# Autodesk Inventor assembly: rapoukMotherboardAssemblyv0
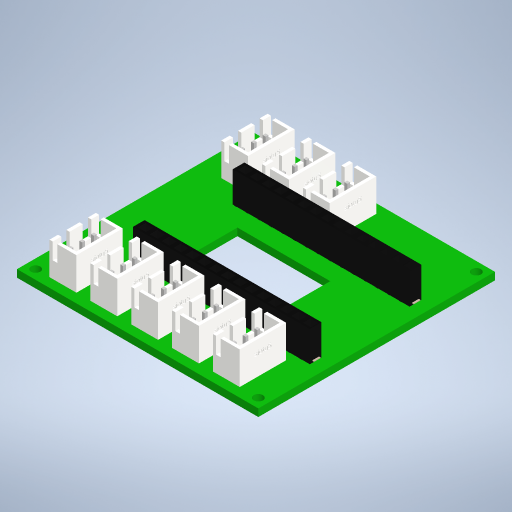
[picture p0: Inventor's stored thumbnail of the model, 512x512]
Saved by Autodesk Inventor 2024 (Build 280153000, 153)
## iProperties
Created: 2024-02-03
Part Number: rapoukMotherboardAssemblyv0
Document SubType Name: Assembly
Designer: Roman Suk
Author: Roman Suk
## Documents named in this file (4)
- C:\Users\Roman Suk\Documents\Ročníkovka SŠ\Technical documentation\Final1\rapoukMotherboardAssemblyv0.iam
- C:\Users\Roman Suk\Documents\Ročníkovka SŠ\Technical documentation\Final1\rapoukMotherboardConnectorv0.ipt
- C:\Users\Roman Suk\Documents\Ročníkovka SŠ\Technical documentation\Final1\rapoukMotherboardPinv0.iam
- C:\Users\Roman Suk\Documents\Ročníkovka SŠ\Technical documentation\Final1\jst 1 v4\jst 1 v4.iam
## Components (11 placed, 3 different names)
1. rapoukMotherboardConnectorv0:1 — Flush:1, Flush:2, Mate:11, Mate:12, Mate:13, Mate:14, Mate:15, Mate:16, Mate:17, Mate:18, Flush:4, Flush:5, Flush:6, Flush:7, Flush:9, Flush:10, Flush:11, Flush:13, Flush:14, Flush:15, Flush:17, Mate:26, Mate:27
2. rapoukMotherboardPinv0:1 [sub-assembly] — Flush:16, Flush:17, Mate:26
3. rapoukMotherboardPinv0:2 [sub-assembly] — Flush:1, Flush:2, Flush:16, Mate:27
4. jst 1 v4:1 [sub-assembly] — Mate:15, Flush:4, Mate:19
5. jst 1 v4:2 [sub-assembly] — Mate:17, Flush:10, Mate:24, Flush:13
6. jst 1 v4:3 [sub-assembly] — Mate:16, Flush:6, Mate:20, Mate:21
7. jst 1 v4:4 [sub-assembly] — Mate:18, Flush:14, Mate:25, Flush:15
8. jst 1 v4:5 [sub-assembly] — Mate:14, Flush:11, Mate:23, Mate:24
9. jst 1 v4:6 [sub-assembly] — Mate:13, Flush:9, Mate:23
10. jst 1 v4:7 [sub-assembly] — Mate:12, Flush:7, Mate:21, Mate:25
11. jst 1 v4:8 [sub-assembly] — Mate:11, Flush:5, Mate:19, Mate:20
## Relationships (30: Mate 16, Flush 14)
- Flush:1 (13.5 mm): rapoukMotherboardConnectorv0:1 ↔ rapoukMotherboardPinv0:2
- Flush:2 (11.5 mm): rapoukMotherboardConnectorv0:1 ↔ rapoukMotherboardPinv0:2
- Mate:11: rapoukMotherboardConnectorv0:1 ↔ jst 1 v4:8
- Mate:12: rapoukMotherboardConnectorv0:1 ↔ jst 1 v4:7
- Mate:13: rapoukMotherboardConnectorv0:1 ↔ jst 1 v4:6
- Mate:14: rapoukMotherboardConnectorv0:1 ↔ jst 1 v4:5
- Mate:15: rapoukMotherboardConnectorv0:1 ↔ jst 1 v4:1
- Mate:16: rapoukMotherboardConnectorv0:1 ↔ jst 1 v4:3
- Mate:17: rapoukMotherboardConnectorv0:1 ↔ jst 1 v4:2
- Mate:18: rapoukMotherboardConnectorv0:1 ↔ jst 1 v4:4
- Flush:4 (2 mm): rapoukMotherboardConnectorv0:1 ↔ jst 1 v4:1
- Flush:5 (2 mm): rapoukMotherboardConnectorv0:1 ↔ jst 1 v4:8
- Flush:6 (2 mm): rapoukMotherboardConnectorv0:1 ↔ jst 1 v4:3
- Flush:7 (2 mm): rapoukMotherboardConnectorv0:1 ↔ jst 1 v4:7
- Flush:9 (2 mm): rapoukMotherboardConnectorv0:1 ↔ jst 1 v4:6
- Flush:10 (2 mm): rapoukMotherboardConnectorv0:1 ↔ jst 1 v4:2
- Flush:11 (2 mm): rapoukMotherboardConnectorv0:1 ↔ jst 1 v4:5
- Mate:19 (3 mm): jst 1 v4:1 ↔ jst 1 v4:8
- Mate:20 (3 mm): jst 1 v4:3 ↔ jst 1 v4:8
- Mate:21 (3 mm): jst 1 v4:3 ↔ jst 1 v4:7
- Mate:23 (3 mm): jst 1 v4:5 ↔ jst 1 v4:6
- Mate:24 (3 mm): jst 1 v4:2 ↔ jst 1 v4:5
- Flush:13 (-5 mm): rapoukMotherboardConnectorv0:1 ↔ jst 1 v4:2
- Flush:14 (2 mm): rapoukMotherboardConnectorv0:1 ↔ jst 1 v4:4
- Mate:25 (3 mm): jst 1 v4:4 ↔ jst 1 v4:7
- Flush:15 (-5 mm): rapoukMotherboardConnectorv0:1 ↔ jst 1 v4:4
- Flush:16: rapoukMotherboardPinv0:1 ↔ rapoukMotherboardPinv0:2
- Flush:17 (-13.5 mm): rapoukMotherboardConnectorv0:1 ↔ rapoukMotherboardPinv0:1
- Mate:26: rapoukMotherboardConnectorv0:1 ↔ rapoukMotherboardPinv0:1
- Mate:27: rapoukMotherboardConnectorv0:1 ↔ rapoukMotherboardPinv0:2
